# Autodesk Inventor assembly: AS_GENERAL
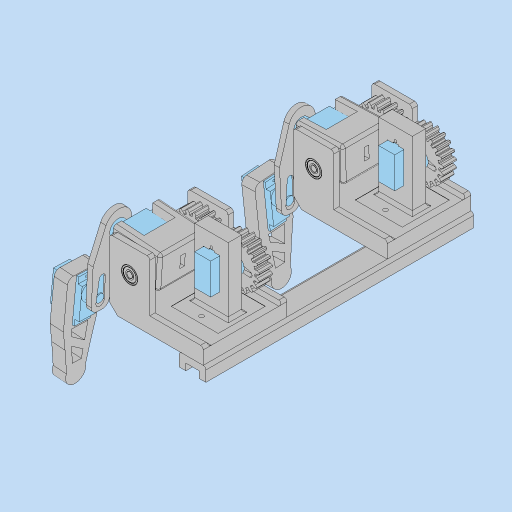
[picture p0: Inventor's stored thumbnail of the model, 512x512]
Saved by Autodesk Inventor 2024 (Build 280153000, 153)
## iProperties
Created: 2024-09-28
Part Number: AS_GENERAL
Document SubType Name: Assembly
Designer: MxMon
Author: MxMon
## Documents named in this file (17)
- C:\Users\MxMon\Documents\Inventor\CHEWIETRON\AS_GENERAL.iam
- C:\Users\MxMon\Documents\Inventor\CHEWIETRON\BASEPRINCIPAL_PATA_IZQ.ipt
- C:\Users\MxMon\Documents\Inventor\CHEWIETRON\bearing_604zz\bearing_604zz.ipt
- C:\Users\MxMon\Documents\Inventor\CHEWIETRON\BASEMOTOR_HOMBRO.ipt
- C:\Users\MxMon\Documents\Inventor\CHEWIETRON\Servo mockup\Servo mockup.ipt
- C:\Users\MxMon\Documents\Inventor\CHEWIETRON\Servo Motor hélice\Servo Motor hélice.ipt
- C:\Users\MxMon\Documents\Inventor\CHEWIETRON\PATA_SUP_IZQ.ipt
- C:\Users\MxMon\Documents\Inventor\CHEWIETRON\PARA_INF.ipt
- C:\Users\MxMon\Documents\Inventor\CHEWIETRON\BASEMOTOR_ENGRANE.ipt
- C:\Users\MxMon\Documents\Inventor\CHEWIETRON\CONECTOR_ENGRANE_HOMBRO.ipt
- C:\Users\MxMon\Documents\Inventor\CHEWIETRON\ENGRANE_HOMBRO.ipt
- C:\Users\MxMon\Documents\Inventor\CHEWIETRON\HELICE_CRUZ.ipt
- C:\Users\MxMon\Documents\Inventor\CHEWIETRON\ENGRANE_HELICE.ipt
- C:\Users\MxMon\Documents\Inventor\CHEWIETRON\EJE_TORNILLO.ipt
- C:\Users\MxMon\Documents\Inventor\CHEWIETRON\TUERCA.ipt
- C:\Users\MxMon\Documents\Inventor\CHEWIETRON\ESPACIADOR.ipt
- C:\Users\MxMon\Documents\Inventor\CHEWIETRON\BASE_DE_PRUEBA.ipt
## Components (39 placed, 16 different names)
1. BASEPRINCIPAL_PATA_IZQ:1 — Mate:1, Mate:2, Mate:3, Mate:4, Mate:23, Mate:25, Mate:46, Mate:98
2. bearing_604zz:1 — Mate:1, Mate:2, Mate:5, Mate:39, Mate:40
3. bearing_604zz:2 — Mate:3, Mate:4, Mate:44
4. BASEMOTOR_HOMBRO:1 — Mate:5, Mate:6, Mate:7, Mate:8, Mate:26, Mate:27, Mate:28, Mate:42
5. Servo mockup:1 — Mate:6, Mate:7, Mate:8, Mate:9, Mate:10
6. Servo Motor hélice:1 — Mate:9, Mate:10, Mate:11, Mate:12, Mate:13
7. PATA_SUP_IZQ:1 — Mate:11, Mate:12, Mate:13, Mate:47, Mate:48, Mate:49, Mate:50
8. Servo mockup:2 — Mate:20, Mate:21, Mate:22
9. Servo Motor hélice:2 — Mate:47, Mate:48, Mate:49, Mate:50
10. PARA_INF:1 — Mate:20, Mate:21, Mate:22
11. BASEMOTOR_ENGRANE:1 — Mate:23, Mate:25, Mate:36, Mate:37, Mate:38, Mate:46
12. CONECTOR_ENGRANE_HOMBRO:1 — Mate:26, Mate:27, Mate:28, Mate:29, Mate:30, Mate:31
13. ENGRANE_HOMBRO:1 — Mate:29, Mate:30, Mate:31
14. Servo mockup:3 — Mate:32, Mate:33, Mate:36, Mate:37, Mate:38
15. HELICE_CRUZ:1 — Mate:32, Mate:33, Mate:34, Mate:35
16. ENGRANE_HELICE:1 — Mate:34, Mate:35
17. EJE_TORNILLO:1 — Mate:39, Mate:40, Mate:41, Mate:43
18. TUERCA:1 — Mate:41, Mate:42, Mate:45
19. ESPACIADOR:1 — Mate:43, Mate:44, Mate:45
20. BASEPRINCIPAL_PATA_IZQ:2 — Mate:97, Mate:99
21. bearing_604zz:3
22. bearing_604zz:4
23. BASEMOTOR_HOMBRO:2
24. Servo mockup:4
25. Servo Motor hélice:3
26. PATA_SUP_IZQ:2
27. Servo mockup:5
28. Servo Motor hélice:4
29. PARA_INF:2
30. BASEMOTOR_ENGRANE:2
31. CONECTOR_ENGRANE_HOMBRO:2
32. ENGRANE_HOMBRO:2
33. Servo mockup:6
34. HELICE_CRUZ:2
35. ENGRANE_HELICE:2
36. EJE_TORNILLO:2
37. TUERCA:2
38. ESPACIADOR:2
39. BASE_DE_PRUEBA:1 — Mate:97, Mate:98, Mate:99
## Relationships (93: Mate 93)
- Mate:1: BASEPRINCIPAL_PATA_IZQ:1 ↔ bearing_604zz:1
- Mate:2: BASEPRINCIPAL_PATA_IZQ:1 ↔ bearing_604zz:1
- Mate:3: BASEPRINCIPAL_PATA_IZQ:1 ↔ bearing_604zz:2
- Mate:4: BASEPRINCIPAL_PATA_IZQ:1 ↔ bearing_604zz:2
- Mate:5: bearing_604zz:1 ↔ BASEMOTOR_HOMBRO:1
- Mate:6: BASEMOTOR_HOMBRO:1 ↔ Servo mockup:1
- Mate:7: BASEMOTOR_HOMBRO:1 ↔ Servo mockup:1
- Mate:8: BASEMOTOR_HOMBRO:1 ↔ Servo mockup:1
- Mate:9: Servo mockup:1 ↔ Servo Motor hélice:1
- Mate:10: Servo mockup:1 ↔ Servo Motor hélice:1
- Mate:11: Servo Motor hélice:1 ↔ PATA_SUP_IZQ:1
- Mate:12: Servo Motor hélice:1 ↔ PATA_SUP_IZQ:1
- Mate:13: Servo Motor hélice:1 ↔ PATA_SUP_IZQ:1
- [Mate]: Servo mockup:2 ↔ Servo Motor hélice:2
- [Mate]: Servo mockup:2 ↔ Servo Motor hélice:2
- Mate:20: Servo mockup:2 ↔ PARA_INF:1
- Mate:21: Servo mockup:2 ↔ PARA_INF:1
- Mate:22: Servo mockup:2 ↔ PARA_INF:1
- Mate:23: BASEPRINCIPAL_PATA_IZQ:1 ↔ BASEMOTOR_ENGRANE:1
- Mate:25: BASEPRINCIPAL_PATA_IZQ:1 ↔ BASEMOTOR_ENGRANE:1
- Mate:26: BASEMOTOR_HOMBRO:1 ↔ CONECTOR_ENGRANE_HOMBRO:1
- Mate:27: BASEMOTOR_HOMBRO:1 ↔ CONECTOR_ENGRANE_HOMBRO:1
- Mate:28: BASEMOTOR_HOMBRO:1 ↔ CONECTOR_ENGRANE_HOMBRO:1
- Mate:29: CONECTOR_ENGRANE_HOMBRO:1 ↔ ENGRANE_HOMBRO:1
- Mate:30: CONECTOR_ENGRANE_HOMBRO:1 ↔ ENGRANE_HOMBRO:1
- Mate:31: CONECTOR_ENGRANE_HOMBRO:1 ↔ ENGRANE_HOMBRO:1
- Mate:32: Servo mockup:3 ↔ HELICE_CRUZ:1
- Mate:33: Servo mockup:3 ↔ HELICE_CRUZ:1
- Mate:34: HELICE_CRUZ:1 ↔ ENGRANE_HELICE:1
- Mate:35: HELICE_CRUZ:1 ↔ ENGRANE_HELICE:1
- Mate:36: BASEMOTOR_ENGRANE:1 ↔ Servo mockup:3
- Mate:37: BASEMOTOR_ENGRANE:1 ↔ Servo mockup:3
- Mate:38: BASEMOTOR_ENGRANE:1 ↔ Servo mockup:3
- Mate:39: bearing_604zz:1 ↔ EJE_TORNILLO:1
- Mate:40: bearing_604zz:1 ↔ EJE_TORNILLO:1
- Mate:41: EJE_TORNILLO:1 ↔ TUERCA:1
- Mate:42: BASEMOTOR_HOMBRO:1 ↔ TUERCA:1
- Mate:43: EJE_TORNILLO:1 ↔ ESPACIADOR:1
- Mate:44: bearing_604zz:2 ↔ ESPACIADOR:1
- Mate:45: TUERCA:1 ↔ ESPACIADOR:1
- Mate:46: BASEPRINCIPAL_PATA_IZQ:1 ↔ BASEMOTOR_ENGRANE:1
- Mate:47: PATA_SUP_IZQ:1 ↔ Servo Motor hélice:2
- Mate:48: PATA_SUP_IZQ:1 ↔ Servo Motor hélice:2
- Mate:49: PATA_SUP_IZQ:1 ↔ Servo Motor hélice:2
- Mate:50: PATA_SUP_IZQ:1 ↔ Servo Motor hélice:2
- [Mate]: BASEPRINCIPAL_PATA_IZQ:2 ↔ bearing_604zz:3
- [Mate]: BASEPRINCIPAL_PATA_IZQ:2 ↔ bearing_604zz:3
- [Mate]: BASEPRINCIPAL_PATA_IZQ:2 ↔ bearing_604zz:4
- [Mate]: BASEPRINCIPAL_PATA_IZQ:2 ↔ bearing_604zz:4
- [Mate]: bearing_604zz:3 ↔ BASEMOTOR_HOMBRO:2
- [Mate]: BASEMOTOR_HOMBRO:2 ↔ Servo mockup:4
- [Mate]: BASEMOTOR_HOMBRO:2 ↔ Servo mockup:4
- [Mate]: BASEMOTOR_HOMBRO:2 ↔ Servo mockup:4
- [Mate]: Servo mockup:4 ↔ Servo Motor hélice:3
- [Mate]: Servo mockup:4 ↔ Servo Motor hélice:3
- [Mate]: Servo Motor hélice:3 ↔ PATA_SUP_IZQ:2
- [Mate]: Servo Motor hélice:3 ↔ PATA_SUP_IZQ:2
- [Mate]: Servo Motor hélice:3 ↔ PATA_SUP_IZQ:2
- [Mate]: Servo mockup:5 ↔ Servo Motor hélice:4
- [Mate]: Servo mockup:5 ↔ Servo Motor hélice:4
- [Mate]: Servo mockup:5 ↔ PARA_INF:2
- [Mate]: Servo mockup:5 ↔ PARA_INF:2
- [Mate]: Servo mockup:5 ↔ PARA_INF:2
- [Mate]: BASEPRINCIPAL_PATA_IZQ:2 ↔ BASEMOTOR_ENGRANE:2
- [Mate]: BASEPRINCIPAL_PATA_IZQ:2 ↔ BASEMOTOR_ENGRANE:2
- [Mate]: BASEMOTOR_HOMBRO:2 ↔ CONECTOR_ENGRANE_HOMBRO:2
- [Mate]: BASEMOTOR_HOMBRO:2 ↔ CONECTOR_ENGRANE_HOMBRO:2
- [Mate]: BASEMOTOR_HOMBRO:2 ↔ CONECTOR_ENGRANE_HOMBRO:2
- [Mate]: CONECTOR_ENGRANE_HOMBRO:2 ↔ ENGRANE_HOMBRO:2
- [Mate]: CONECTOR_ENGRANE_HOMBRO:2 ↔ ENGRANE_HOMBRO:2
- [Mate]: CONECTOR_ENGRANE_HOMBRO:2 ↔ ENGRANE_HOMBRO:2
- [Mate]: Servo mockup:6 ↔ HELICE_CRUZ:2
- [Mate]: Servo mockup:6 ↔ HELICE_CRUZ:2
- [Mate]: HELICE_CRUZ:2 ↔ ENGRANE_HELICE:2
- [Mate]: HELICE_CRUZ:2 ↔ ENGRANE_HELICE:2
- [Mate]: BASEMOTOR_ENGRANE:2 ↔ Servo mockup:6
- [Mate]: BASEMOTOR_ENGRANE:2 ↔ Servo mockup:6
- [Mate]: BASEMOTOR_ENGRANE:2 ↔ Servo mockup:6
- [Mate]: bearing_604zz:3 ↔ EJE_TORNILLO:2
- [Mate]: bearing_604zz:3 ↔ EJE_TORNILLO:2
- [Mate]: EJE_TORNILLO:2 ↔ TUERCA:2
- [Mate]: BASEMOTOR_HOMBRO:2 ↔ TUERCA:2
- [Mate]: EJE_TORNILLO:2 ↔ ESPACIADOR:2
- [Mate]: bearing_604zz:4 ↔ ESPACIADOR:2
- [Mate]: TUERCA:2 ↔ ESPACIADOR:2
- [Mate]: BASEPRINCIPAL_PATA_IZQ:2 ↔ BASEMOTOR_ENGRANE:2
- [Mate]: PATA_SUP_IZQ:2 ↔ Servo Motor hélice:4
- [Mate]: PATA_SUP_IZQ:2 ↔ Servo Motor hélice:4
- [Mate]: PATA_SUP_IZQ:2 ↔ Servo Motor hélice:4
- [Mate]: PATA_SUP_IZQ:2 ↔ Servo Motor hélice:4
- Mate:97: BASEPRINCIPAL_PATA_IZQ:2 ↔ BASE_DE_PRUEBA:1
- Mate:98: BASEPRINCIPAL_PATA_IZQ:1 ↔ BASE_DE_PRUEBA:1
- Mate:99: BASEPRINCIPAL_PATA_IZQ:2 ↔ BASE_DE_PRUEBA:1
## Named parameters: d16_d8 = 0 mm, d17_d9 = 0 mm, d57_d0 = 0 mm, d58_d1 = 0 mm, d59_d2 = 0 mm, d60_d3 = 0 mm, d61_d4 = 0 mm, d62_d5 = 0 mm, d63_d6 = 0 mm, d64_d7 = 0 mm, d65_d8 = 0 mm, d66_d9 = 0 mm, d67_d12 = 0 mm, d68_d24 = 0 mm, d69_d25 = 0 mm, d70_d26 = 0 mm, d71_d27 = 0 mm, d72_d29 = 0 mm, d73_d30 = 0 mm, d74_d31 = 0 mm, d75_d32 = 0 mm, d76_d33 = 0 mm, d77_d34 = 0 mm, d78_d35 = 0 mm, d79_d14 = 0 mm, d80_d15 = 0 mm, d81_d16_d8 = 0 mm, d82_d17_d9 = 0 mm, d83_d36 = 0 mm, d84_d37 = 0 mm, d85_d38 = 0 mm, d86_d39 = 0 mm, d87_d40 = 0 mm, d88_d41 = 0 mm, d89_d42 = 0 mm, d90_d43 = 0 mm, d91_d44 = 0 mm, d92_d45 = 0 mm, d93_d46 = 0 mm, d94_d47 = 0 mm, d95_d48 = 0 mm, d96_d49 = 0 mm, d97_d50 = 0 mm, d98_d51 = 0 mm, d99_d53 = 0 mm, d100_d54 = 0 mm, d101_d55 = 0 mm
